# Autodesk Inventor assembly: mill_assembly
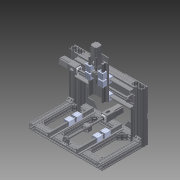
[picture p0: Inventor's stored thumbnail of the model, 180x180]
Saved by Autodesk Inventor 2014 (Build 180170000, 170)
## iProperties
Created: 2014-08-08
Part Number: mill_assembly
Document SubType Name: Assembly
Designer: Matthew
Author: Matthew
## Documents named in this file (34)
- C:\Users\Matthew\Documents\GitHub\CNC Mill\mill_assembly.iam
- C:\Users\Matthew\Documents\GitHub\CNC Mill\8020\2020.ipt
- C:\Users\Matthew\Documents\GitHub\CNC Mill\8020\2020_18in.ipt
- C:\Users\Matthew\Documents\GitHub\CNC Mill\8020\gusset_4138.ipt
- C:\Users\Matthew\Documents\GitHub\CNC Mill\8020\gusset_4134.ipt
- C:\Users\Matthew\Documents\GitHub\CNC Mill\mic6_plate.ipt
- C:\Users\Matthew\Documents\GitHub\CNC Mill\1605\1605_400mm.ipt
- C:\Users\Matthew\Documents\GitHub\CNC Mill\1605\1605_ballnut.ipt
- C:\Users\Matthew\Documents\GitHub\CNC Mill\nema23_motor_mount.ipt
- C:\Users\Matthew\Documents\GitHub\CNC Mill\fk12.ipt
- C:\Users\Matthew\Documents\GitHub\CNC Mill\sbr\sbr20\SBR20UU.iam
- C:\Users\Matthew\Documents\GitHub\CNC Mill\6.35x10mm_coupler.ipt
- C:\Users\Matthew\Documents\GitHub\CNC Mill\sbr\sbr20\sbr20_400mm.ipt
- C:\Users\Matthew\Documents\GitHub\CNC Mill\HD16.ipt
- C:\Users\Matthew\Documents\GitHub\CNC Mill\nema23_HS8630.ipt
- C:\Users\Matthew\Documents\GitHub\CNC Mill\z-axis_mount_plate.ipt
- C:\Users\Matthew\Documents\GitHub\CNC Mill\1605\1605_200mm.ipt
- C:\Users\Matthew\Documents\GitHub\CNC Mill\y-axis_mount_plate.ipt
- C:\Users\Matthew\Documents\GitHub\CNC Mill\router_plate.ipt
- C:\Users\Matthew\Documents\GitHub\CNC Mill\router_mount.ipt
- C:\Users\Matthew\Documents\GitHub\CNC Mill\1617evs.ipt
- C:\Users\Matthew\Documents\GitHub\CNC Mill\ff12_mount.ipt
- C:\Users\Matthew\Documents\GitHub\CNC Mill\ff12.ipt
- C:\Users\Matthew\Documents\GitHub\CNC Mill\sbr\sbr20\sbr20_500mm.ipt
- C:\Users\Matthew\Documents\GitHub\CNC Mill\1605\1605_500mm.ipt
- C:\Users\Matthew\Documents\GitHub\CNC Mill\sbr\sbr20\sbr20_300mm.ipt
- C:\Users\Matthew\Documents\GitHub\CNC Mill\8020\2040_top_bar.ipt
- C:\Users\Matthew\Documents\GitHub\CNC Mill\8020\2040_uprights.ipt
- C:\Users\Matthew\Downloads\Imported Components\endmill 2 flute_finishing\endmill 2 flute_finishing.ipt
- C:\Users\Matthew\Downloads\Imported Components\User Library-ER COLLET\Assembly1.iam
- C:\Users\Matthew\Documents\GitHub\CNC Mill\8020\2020_rear.ipt
- C:\Users\Matthew\Documents\GitHub\CNC Mill\8020\2020_front.ipt
- C:\Users\Matthew\Documents\GitHub\CNC Mill\8020\2040-2040_mounting_plate.ipt
- C:\Users\Matthew\Documents\GitHub\CNC Mill\8020\2020-2040_mounting_plate.ipt
## Components (80 placed, 33 different names)
1. 2020_18in:1 — Mate:31, Mate:32, Mate:38, Mate:47, Mate:48, Flush:161, Flush:168, Mate:253
2. 2020_18in:2 — Mate:28, Mate:29, Mate:34, Mate:50, Mate:51, Mate:241, Flush:163, Mate:242, Flush:164, Mate:255, Flush:171, Flush:172
3. gusset_4138:1 — Mate:260, Mate:261, Flush:175
4. gusset_4134:1 — Mate:28, Mate:29, Mate:275
5. gusset_4138:2 — Mate:258, Mate:259, Mate:262, Flush:175
6. gusset_4134:2 — Mate:31, Mate:32, Mate:276
7. gusset_4134:3 — Mate:34, Flush:61, Flush:147, Mate:278
8. gusset_4134:4 — Mate:38, Flush:62, Flush:153, Mate:279
9. gusset_4134:5 — Mate:50, Mate:51, Flush:148, Flush:188
10. gusset_4134:6 — Mate:47, Mate:48, Flush:61, Flush:62, Mate:269, Flush:186
11. mic6_plate:1 — Flush:76, Flush:77, Mate:141
12. 1605_400mm:1 — Mate:98, Mate:100, Mate:108, Insert:2, Insert:13
13. 1605_ballnut:1 — Mate:108, Mate:133, Mate:134, Flush:75
14. nema23_motor_mount:1 — Mate:99, Mate:136, Mate:137, Mate:254
15. nema23_motor_mount:2 — Mate:153, Flush:86, Mate:154, Mate:155, Mate:156, Mate:157
16. 1605_ballnut:6 — Mate:150, Mate:158, Flush:90, Mate:159
17. fk12:1 — Mate:98, Mate:99, Mate:100, Mate:137, Mate:217
18. fk12:3 — Mate:156, Mate:157, Mate:214
19. SBR20UU:1 [sub-assembly] — Mate:131, Flush:69, Flush:70, Flush:73, Mate:138, Mate:140, Flush:77, Mate:141
20. 6.35x10mm_coupler:1 — Insert:3, Insert:4
21. sbr20_400mm:1 — Mate:130, Flush:136, Mate:217, Mate:247, Flush:191
22. SBR20UU:2 [sub-assembly] — Mate:129, Mate:132, Flush:71, Flush:72, Mate:139
23. sbr20_400mm:2 — Mate:129, Flush:136, Mate:248, Flush:190
24. SBR20UU:3 [sub-assembly] — Mate:130, Mate:131, Flush:69, Flush:70, Flush:74, Flush:76, Mate:274
25. SBR20UU:4 [sub-assembly] — Mate:132, Flush:71, Flush:72, Flush:73, Flush:74
26. HD16:1 — Mate:133, Mate:134, Flush:75, Mate:138, Mate:139, Mate:140, Mate:274
27. nema23_HS8630:1 — Mate:135, Mate:136
28. 6.35x10mm_coupler:2 — Insert:2, Mate:135
29. SBR20UU:5 [sub-assembly] — Flush:78, Flush:79, Mate:144, Flush:84, Flush:85, Mate:160
30. SBR20UU:6 [sub-assembly] — Flush:78, Flush:79, Mate:144, Mate:213
31. SBR20UU:7 [sub-assembly] — Flush:84, Flush:85
32. SBR20UU:8 [sub-assembly] — Mate:212
33. z-axis_mount_plate:1 — Mate:153, Flush:86, Mate:167, Flush:102, Flush:103, Mate:208, Mate:209, Flush:139
34. 1605_200mm:1 — Mate:150, Insert:3
35. nema23_HS8630:2 — Mate:154, Mate:155, Insert:4
36. HD16:6 — Mate:158, Flush:90, Mate:159, Mate:160, Mate:186, Flush:120, Flush:121, Mate:210, Mate:211
37. y-axis_mount_plate:1 — Mate:177, Mate:199, Mate:200, Flush:135, Mate:206, Flush:137, Flush:184, Mate:267, Flush:185
38. SBR20UU:9 [sub-assembly] — Flush:95, Flush:96, Flush:99, Flush:101, Mate:167, Flush:103, Mate:201
39. SBR20UU:10 [sub-assembly] — Flush:95, Flush:96, Mate:166, Flush:97, Flush:98, Flush:102
40. SBR20UU:11 [sub-assembly] — Flush:99, Flush:100, Flush:101
41. SBR20UU:12 [sub-assembly] — Mate:166, Flush:97, Flush:98, Flush:100, Mate:180, Mate:202
42. nema23_motor_mount:4 — Mate:177, Flush:137
43. fk12:4 — Mate:204, Insert:10
44. 6.35x10mm_coupler:3
45. nema23_HS8630:3
46. 1605_ballnut:7 — Mate:240
47. HD16:7 — Mate:180, Mate:203, Mate:205
48. router_plate:1 — Mate:186, Flush:120, Flush:121, Mate:187, Flush:122, Flush:123
49. router_mount:1 — Insert:7, Mate:187, Flush:122, Flush:123
50. 1617evs:1 — Insert:7
51. ff12_mount:1 — Insert:9, Mate:256
52. ff12:1 — Insert:9, Insert:13
53. sbr20_500mm:1 — Flush:133, Mate:200, Mate:201, Mate:203, Mate:204, Flush:135
54. sbr20_500mm:2 — Flush:133, Mate:199, Mate:202, Mate:205
55. 1605_500mm:1 — Insert:10, Insert:11, Mate:240
56. ff12:2 — Insert:11, Insert:12
57. ff12_mount:2 — Insert:12, Mate:206
58. sbr20_300mm:1 — Flush:138, Mate:208, Mate:210, Mate:213, Mate:214, Flush:139
59. sbr20_300mm:2 — Flush:138, Mate:209, Mate:211, Mate:212
60. 2020:1 — Mate:223, Mate:230, Mate:233, Mate:248, Mate:250, Flush:169, Mate:271, Flush:190
61. 2020:2 — Mate:222, Mate:224, Mate:226, Mate:247, Mate:251, Flush:170, Mate:273, Flush:191
62. gusset_4134:8 — Mate:222, Flush:147, Mate:277
63. gusset_4134:9 — Mate:223, Flush:148, Flush:149, Flush:150, Flush:151, Mate:280
64. gusset_4134:11 — Mate:224, Flush:149, Mate:268
65. gusset_4134:12 — Mate:230, Flush:151
66. gusset_4134:13 — Mate:226, Flush:150, Mate:281
67. gusset_4134:14 — Flush:153, Mate:233
68. 2040_top_bar:1 — Mate:257, Flush:173, Flush:174, Mate:258, Mate:261, Flush:176, Mate:264, Flush:184, Mate:267
69. 2040_uprights:1 — Flush:161, Mate:241, Flush:167, Mate:252, Flush:168, Mate:253, Mate:257, Flush:173, Flush:174, Mate:259, Mate:262, Flush:177, Mate:263, Mate:266, Flush:182, Flush:185, Mate:269, Flush:187, Mate:276
70. endmill 2 flute_finishing:1
71. Assembly1:1 [sub-assembly]
72. 2040_uprights:2 — Flush:163, Mate:242, Flush:164, Mate:249, Flush:165, Flush:166, Mate:260, Flush:178, Flush:179, Mate:265, Flush:181, Flush:189, Mate:275
73. 2020_rear:1 — Mate:249, Flush:165, Flush:166, Mate:250, Mate:251, Flush:167, Mate:252, Flush:169, Flush:170, Mate:254, Flush:180, Flush:183, Mate:268, Mate:270, Mate:272, Mate:280
74. 2020_front:1 — Mate:255, Flush:171, Flush:172, Mate:256, Mate:277, Mate:278, Mate:279, Mate:281
75. 2040-2040_mounting_plate:1 — Flush:176, Flush:177, Mate:263
76. 2040-2040_mounting_plate:2 — Mate:264, Flush:178, Flush:179
77. 2020-2040_mounting_plate:1 — Mate:265, Flush:180, Flush:181
78. 2020-2040_mounting_plate:2 — Mate:266, Flush:182, Flush:183
79. gusset_4138:3 — Mate:270, Flush:186, Flush:187, Mate:271
80. gusset_4138:4 — Mate:272, Flush:188, Flush:189, Mate:273
## Relationships (195: Mate 110, Flush 75, Insert 10)
- Mate:28: 2020_18in:2 ↔ gusset_4134:1
- Mate:29: 2020_18in:2 ↔ gusset_4134:1
- Mate:31: 2020_18in:1 ↔ gusset_4134:2
- Mate:32: 2020_18in:1 ↔ gusset_4134:2
- Mate:34: 2020_18in:2 ↔ gusset_4134:3
- Mate:38: 2020_18in:1 ↔ gusset_4134:4
- Mate:47: 2020_18in:1 ↔ gusset_4134:6
- Mate:48: 2020_18in:1 ↔ gusset_4134:6
- Mate:50: 2020_18in:2 ↔ gusset_4134:5
- Mate:51: 2020_18in:2 ↔ gusset_4134:5
- Mate:98: 1605_400mm:1 ↔ fk12:1
- Mate:99: nema23_motor_mount:1 ↔ fk12:1
- Mate:100: 1605_400mm:1 ↔ fk12:1
- Mate:108: 1605_400mm:1 ↔ 1605_ballnut:1
- Flush:61: gusset_4134:3 ↔ gusset_4134:6
- Flush:62: gusset_4134:4 ↔ gusset_4134:6
- Mate:129: SBR20UU:2 ↔ sbr20_400mm:2
- Mate:130: sbr20_400mm:1 ↔ SBR20UU:3
- Mate:131 (20 mm): SBR20UU:1 ↔ SBR20UU:3
- Flush:69: SBR20UU:1 ↔ SBR20UU:3
- Flush:70: SBR20UU:1 ↔ SBR20UU:3
- Mate:132 (20 mm): SBR20UU:2 ↔ SBR20UU:4
- Flush:71: SBR20UU:2 ↔ SBR20UU:4
- Flush:72: SBR20UU:2 ↔ SBR20UU:4
- Flush:73: SBR20UU:1 ↔ SBR20UU:4
- Flush:74: SBR20UU:3 ↔ SBR20UU:4
- Mate:133: 1605_ballnut:1 ↔ HD16:1
- Mate:134: 1605_ballnut:1 ↔ HD16:1
- Flush:75: 1605_ballnut:1 ↔ HD16:1
- Insert:2 (-12.5 mm): 1605_400mm:1 ↔ 6.35x10mm_coupler:2
- Mate:135: nema23_HS8630:1 ↔ 6.35x10mm_coupler:2
- Mate:136: nema23_motor_mount:1 ↔ nema23_HS8630:1
- Mate:137: nema23_motor_mount:1 ↔ fk12:1
- Mate:138 (93.1 mm): SBR20UU:1 ↔ HD16:1
- Mate:139 (93.1 mm): SBR20UU:2 ↔ HD16:1
- Mate:140 (-7.5 mm): SBR20UU:1 ↔ HD16:1
- Flush:76 (52.6255 mm): mic6_plate:1 ↔ SBR20UU:3
- Flush:77 (-92.4052 mm): mic6_plate:1 ↔ SBR20UU:1
- Mate:141: mic6_plate:1 ↔ SBR20UU:1
- Flush:78: SBR20UU:5 ↔ SBR20UU:6
- Flush:79: SBR20UU:5 ↔ SBR20UU:6
- Mate:144 (10 mm): SBR20UU:5 ↔ SBR20UU:6
- [Flush]: SBR20UU:7 ↔ SBR20UU:8
- [Flush]: SBR20UU:7 ↔ SBR20UU:8
- [Mate] (10 mm): SBR20UU:7 ↔ SBR20UU:8
- Flush:84: SBR20UU:5 ↔ SBR20UU:7
- Flush:85: SBR20UU:5 ↔ SBR20UU:7
- Mate:150: 1605_ballnut:6 ↔ 1605_200mm:1
- Insert:3 (-12.5 mm): 6.35x10mm_coupler:1 ↔ 1605_200mm:1
- Mate:153: nema23_motor_mount:2 ↔ z-axis_mount_plate:1
- Flush:86: nema23_motor_mount:2 ↔ z-axis_mount_plate:1
- Mate:154: nema23_motor_mount:2 ↔ nema23_HS8630:2
- Mate:155: nema23_motor_mount:2 ↔ nema23_HS8630:2
- Insert:4 (-7 mm): 6.35x10mm_coupler:1 ↔ nema23_HS8630:2
- Mate:156: nema23_motor_mount:2 ↔ fk12:3
- Mate:157: nema23_motor_mount:2 ↔ fk12:3
- Mate:158: 1605_ballnut:6 ↔ HD16:6
- Flush:90: 1605_ballnut:6 ↔ HD16:6
- Mate:159: 1605_ballnut:6 ↔ HD16:6
- Mate:160 (-12.5 mm): SBR20UU:5 ↔ HD16:6
- Flush:95: SBR20UU:9 ↔ SBR20UU:10
- Flush:96: SBR20UU:9 ↔ SBR20UU:10
- Mate:166 (60 mm): SBR20UU:10 ↔ SBR20UU:12
- Flush:97: SBR20UU:10 ↔ SBR20UU:12
- Flush:98: SBR20UU:10 ↔ SBR20UU:12
- Flush:99: SBR20UU:9 ↔ SBR20UU:11
- Flush:100: SBR20UU:11 ↔ SBR20UU:12
- Flush:101: SBR20UU:9 ↔ SBR20UU:11
- Mate:167: z-axis_mount_plate:1 ↔ SBR20UU:9
- Flush:102: z-axis_mount_plate:1 ↔ SBR20UU:10
- Flush:103: z-axis_mount_plate:1 ↔ SBR20UU:9
- [Mate]: nema23_motor_mount:4 ↔ nema23_HS8630:3
- [Mate]: nema23_motor_mount:4 ↔ nema23_HS8630:3
- [Insert] (-7 mm): 6.35x10mm_coupler:3 ↔ nema23_HS8630:3
- [Mate]: nema23_motor_mount:4 ↔ fk12:4
- [Mate]: nema23_motor_mount:4 ↔ fk12:4
- [Mate]: 1605_ballnut:7 ↔ HD16:7
- [Flush]: 1605_ballnut:7 ↔ HD16:7
- [Mate]: 1605_ballnut:7 ↔ HD16:7
- Mate:177: y-axis_mount_plate:1 ↔ nema23_motor_mount:4
- Mate:180 (12.5 mm): SBR20UU:12 ↔ HD16:7
- Insert:7: router_mount:1 ↔ 1617evs:1
- Mate:186: HD16:6 ↔ router_plate:1
- Flush:120 (-96.7994 mm): HD16:6 ↔ router_plate:1
- Flush:121 (64.897 mm): HD16:6 ↔ router_plate:1
- Mate:187: router_plate:1 ↔ router_mount:1
- Flush:122: router_plate:1 ↔ router_mount:1
- Flush:123 (44.45 mm): router_plate:1 ↔ router_mount:1
- Insert:9: ff12_mount:1 ↔ ff12:1
- Flush:133: sbr20_500mm:1 ↔ sbr20_500mm:2
- Mate:199: y-axis_mount_plate:1 ↔ sbr20_500mm:2
- Mate:200: y-axis_mount_plate:1 ↔ sbr20_500mm:1
- Mate:201: SBR20UU:9 ↔ sbr20_500mm:1
- Mate:202: SBR20UU:12 ↔ sbr20_500mm:2
- Mate:203 (19.9 mm): HD16:7 ↔ sbr20_500mm:1
- Mate:204 (-40 mm): fk12:4 ↔ sbr20_500mm:1
- Mate:205 (19.9 mm): HD16:7 ↔ sbr20_500mm:2
- Flush:135: y-axis_mount_plate:1 ↔ sbr20_500mm:1
- Flush:136: sbr20_400mm:1 ↔ sbr20_400mm:2
- Insert:10: fk12:4 ↔ 1605_500mm:1
- Insert:11: 1605_500mm:1 ↔ ff12:2
- Insert:12: ff12:2 ↔ ff12_mount:2
- Mate:206: y-axis_mount_plate:1 ↔ ff12_mount:2
- Insert:13: 1605_400mm:1 ↔ ff12:1
- Flush:137: y-axis_mount_plate:1 ↔ nema23_motor_mount:4
- Flush:138: sbr20_300mm:1 ↔ sbr20_300mm:2
- Mate:208: z-axis_mount_plate:1 ↔ sbr20_300mm:1
- Mate:209: z-axis_mount_plate:1 ↔ sbr20_300mm:2
- Mate:210 (11 mm): HD16:6 ↔ sbr20_300mm:1
- Mate:211 (11 mm): HD16:6 ↔ sbr20_300mm:2
- Mate:212: SBR20UU:8 ↔ sbr20_300mm:2
- Mate:213: SBR20UU:6 ↔ sbr20_300mm:1
- Mate:214 (-40 mm): fk12:3 ↔ sbr20_300mm:1
- Flush:139: z-axis_mount_plate:1 ↔ sbr20_300mm:1
- Mate:217 (-40 mm): fk12:1 ↔ sbr20_400mm:1
- Mate:222: 2020:2 ↔ gusset_4134:8
- Flush:147: gusset_4134:3 ↔ gusset_4134:8
- Mate:223: 2020:1 ↔ gusset_4134:9
- Mate:224: 2020:2 ↔ gusset_4134:11
- Mate:226: 2020:2 ↔ gusset_4134:13
- Flush:148: gusset_4134:5 ↔ gusset_4134:9
- Flush:149: gusset_4134:9 ↔ gusset_4134:11
- Mate:230: 2020:1 ↔ gusset_4134:12
- Flush:150: gusset_4134:9 ↔ gusset_4134:13
- Flush:151: gusset_4134:9 ↔ gusset_4134:12
- Flush:153: gusset_4134:4 ↔ gusset_4134:14
- Mate:233: 2020:1 ↔ gusset_4134:14
- Mate:240: 1605_ballnut:7 ↔ 1605_500mm:1
- Flush:161: 2020_18in:1 ↔ 2040_uprights:1
- Mate:241: 2020_18in:2 ↔ 2040_uprights:1
- Flush:163: 2020_18in:2 ↔ 2040_uprights:2
- Mate:242: 2020_18in:2 ↔ 2040_uprights:2
- Flush:164: 2020_18in:2 ↔ 2040_uprights:2
- Mate:247: sbr20_400mm:1 ↔ 2020:2
- Mate:248: sbr20_400mm:2 ↔ 2020:1
- Mate:249: 2040_uprights:2 ↔ 2020_rear:1
- Flush:165: 2040_uprights:2 ↔ 2020_rear:1
- Flush:166: 2040_uprights:2 ↔ 2020_rear:1
- Mate:250: 2020:1 ↔ 2020_rear:1
- Mate:251: 2020:2 ↔ 2020_rear:1
- Flush:167: 2040_uprights:1 ↔ 2020_rear:1
- Mate:252: 2040_uprights:1 ↔ 2020_rear:1
- Flush:168: 2020_18in:1 ↔ 2040_uprights:1
- Mate:253: 2020_18in:1 ↔ 2040_uprights:1
- Flush:169: 2020:1 ↔ 2020_rear:1
- Flush:170: 2020:2 ↔ 2020_rear:1
- Mate:254: nema23_motor_mount:1 ↔ 2020_rear:1
- Mate:255: 2020_18in:2 ↔ 2020_front:1
- Flush:171: 2020_18in:2 ↔ 2020_front:1
- Flush:172: 2020_18in:2 ↔ 2020_front:1
- Mate:256: ff12_mount:1 ↔ 2020_front:1
- Mate:257: 2040_top_bar:1 ↔ 2040_uprights:1
- Flush:173: 2040_top_bar:1 ↔ 2040_uprights:1
- Flush:174: 2040_top_bar:1 ↔ 2040_uprights:1
- Mate:258: gusset_4138:2 ↔ 2040_top_bar:1
- Mate:259: gusset_4138:2 ↔ 2040_uprights:1
- Mate:260: gusset_4138:1 ↔ 2040_uprights:2
- Mate:261: gusset_4138:1 ↔ 2040_top_bar:1
- Mate:262: gusset_4138:2 ↔ 2040_uprights:1
- Flush:175: gusset_4138:1 ↔ gusset_4138:2
- Flush:176: 2040_top_bar:1 ↔ 2040-2040_mounting_plate:1
- Flush:177: 2040_uprights:1 ↔ 2040-2040_mounting_plate:1
- Mate:263: 2040_uprights:1 ↔ 2040-2040_mounting_plate:1
- Mate:264: 2040_top_bar:1 ↔ 2040-2040_mounting_plate:2
- Flush:178: 2040_uprights:2 ↔ 2040-2040_mounting_plate:2
- Flush:179: 2040_uprights:2 ↔ 2040-2040_mounting_plate:2
- Mate:265: 2040_uprights:2 ↔ 2020-2040_mounting_plate:1
- Flush:180: 2020_rear:1 ↔ 2020-2040_mounting_plate:1
- Flush:181: 2040_uprights:2 ↔ 2020-2040_mounting_plate:1
- Mate:266: 2040_uprights:1 ↔ 2020-2040_mounting_plate:2
- Flush:182: 2040_uprights:1 ↔ 2020-2040_mounting_plate:2
- Flush:183: 2020_rear:1 ↔ 2020-2040_mounting_plate:2
- Flush:184: y-axis_mount_plate:1 ↔ 2040_top_bar:1
- Mate:267: y-axis_mount_plate:1 ↔ 2040_top_bar:1
- Flush:185 (50.8 mm): y-axis_mount_plate:1 ↔ 2040_uprights:1
- Mate:268: gusset_4134:11 ↔ 2020_rear:1
- Mate:269: gusset_4134:6 ↔ 2040_uprights:1
- Mate:270: 2020_rear:1 ↔ gusset_4138:3
- Flush:186: gusset_4134:6 ↔ gusset_4138:3
- Flush:187 (-76.2 mm): 2040_uprights:1 ↔ gusset_4138:3
- Mate:271: 2020:1 ↔ gusset_4138:3
- Mate:272: 2020_rear:1 ↔ gusset_4138:4
- Flush:188: gusset_4134:5 ↔ gusset_4138:4
- Flush:189 (76.2 mm): 2040_uprights:2 ↔ gusset_4138:4
- Mate:273: 2020:2 ↔ gusset_4138:4
- Flush:190: sbr20_400mm:2 ↔ 2020:1
- Flush:191: sbr20_400mm:1 ↔ 2020:2
- Mate:274 (78.5745 mm): SBR20UU:3 ↔ HD16:1
- Mate:275: gusset_4134:1 ↔ 2040_uprights:2
- Mate:276: gusset_4134:2 ↔ 2040_uprights:1
- Mate:277: gusset_4134:8 ↔ 2020_front:1
- Mate:278: gusset_4134:3 ↔ 2020_front:1
- Mate:279: gusset_4134:4 ↔ 2020_front:1
- Mate:280: gusset_4134:9 ↔ 2020_rear:1
- Mate:281: gusset_4134:13 ↔ 2020_front:1
## Named parameters: mountspace = 20 mm, yoffset = 93.1 mm, d321_d318 = 0 mm, d322_d319 = 0 mm, d323_d320 = 10 mm, yaxisspacing = 60 mm, d373_d340 = -7 mm, d374_d341 = 0 mm, d375_d342 = 0 mm, d376_d338 = 0 mm, d377_d339 = 0 mm, d379_d346 = 0 mm, d380_d347 = 0 mm, d381_d348 = 0 mm, yaxissbrspacing = 19.9 mm, yaxis_spacing = 78.5745 mm
